# Autodesk Inventor assembly: Assembly_SIMMO_1
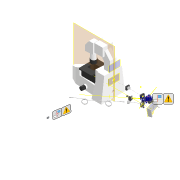
[picture p0: Inventor's stored thumbnail of the model, 180x180]
Saved by Autodesk Inventor 2022 (Build 260153000, 153)
## iProperties
Created: 2022-04-09
Part Number: Assembly_SIMMO_1
Document SubType Name: Assembly
Designer: Prakash Lab
Author: Prakash Lab
## Documents named in this file (16)
- C:\Users\PrakashLab\Documents\SIMMO\INVENTOR\Assembly_SIMMO_1.iam
- C:\Users\PrakashLab\Documents\SIMMO\INVENTOR\00_AC254-200-A-ML-Step.ipt
- C:\Users\PrakashLab\Documents\SIMMO\INVENTOR\Adapter_DMD_KM100.ipt
- C:\Users\PrakashLab\Documents\SIMMO\INVENTOR\Cover_new.ipt
- C:\Users\PrakashLab\Documents\SIMMO\INVENTOR\KM100-Solidworks.ipt
- C:\Users\PrakashLab\Documents\SIMMO\INVENTOR\Mount_new.ipt
- C:\Users\PrakashLab\Documents\SIMMO\INVENTOR\Nikon_Ti2E.ipt
- C:\Users\PrakashLab\Documents\SIMMO\INVENTOR\00_AC254-030-A-ML-Step.ipt
- C:\Users\PrakashLab\Documents\SIMMO\INVENTOR\00_AC254-075-A-ML-Step.ipt
- C:\Users\PrakashLab\Documents\SIMMO\INVENTOR\00_Beampath_v0.ipt
- C:\Users\PrakashLab\Documents\SIMMO\INVENTOR\PF10-03-P01-Solidworks.ipt
- C:\Users\PrakashLab\Documents\SIMMO\INVENTOR\00_Assembly_Axiovert.ipt
- C:\Users\PrakashLab\Documents\SIMMO\INVENTOR\00_CP33T_M-Step.ipt
- C:\Users\PrakashLab\Documents\SIMMO\INVENTOR\00_KM100-Step.ipt
- C:\Users\PrakashLab\Documents\SIMMO\INVENTOR\00_P1-305A-FC-1-Step.ipt
- C:\Users\PrakashLab\Documents\SIMMO\INVENTOR\00_PF10-03-P01-Solidworks.ipt
## Components (19 placed, 15 different names)
1. Adapter_DMD_KM100:1 — Insert:5, Mate:5, Insert:6, Mate:6
2. KM100-Solidworks:1 — Insert:6, Angle:3
3. Mount_new:1 — Mate:6
4. 00_AC254-030-A-ML-Step:1 — Insert:11, Insert:12
5. Nikon_Ti2E:1 — Mate:1, Mate:2, Mate:3, Flush:1, Flush:2, Flush:4, Mate:10, Mate:11, Angle:6
6. 00_Beampath_v0:1 — Flush:1, Flush:2, Insert:1, Insert:2, Insert:3, Angle:1, Mate:4, Angle:4, Mate:7, Mate:8, Mate:12, Insert:12, Insert:13, Insert:15
7. 00_AC254-200-A-ML-Step:1 — Insert:1
8. 00_AC254-075-A-ML-Step:1 — Insert:2, Insert:8
9. 00_AC254-075-A-ML-Step:2 — Insert:3, Insert:9
10. Cover_new:1 — Angle:1, Mate:4, Angle:2, Insert:5, Mate:5
11. PF10-03-P01-Solidworks:1 — Angle:4, Mate:7, Mate:8
12. 00_Assembly_Axiovert:1 — Flush:4, Mate:10, Mate:11, Mate:12
13. 00_CP33T_M-Step:1 — Insert:8
14. 00_CP33T_M-Step:2 — Insert:9
15. 00_KM100-Step:2 — Insert:16
16. 00_P1-305A-FC-1-Step:1 — Insert:11
17. 00_KM100-Step:3 — Insert:14, Angle:6
18. 00_PF10-03-P01-Solidworks:1 — Insert:13, Insert:14
19. 00_PF10-03-P01-Solidworks:2 — Insert:15, Insert:16
## Relationships (32: Insert 13, Mate 11, Angle 5, Flush 3)
- Mate:1: Nikon_Ti2E:1
- Mate:2: Nikon_Ti2E:1
- Mate:3: Nikon_Ti2E:1
- Flush:1: Nikon_Ti2E:1 ↔ 00_Beampath_v0:1
- Flush:2: Nikon_Ti2E:1 ↔ 00_Beampath_v0:1
- Insert:1: 00_Beampath_v0:1 ↔ 00_AC254-200-A-ML-Step:1
- Insert:2: 00_Beampath_v0:1 ↔ 00_AC254-075-A-ML-Step:1
- Insert:3: 00_Beampath_v0:1 ↔ 00_AC254-075-A-ML-Step:2
- Angle:1 (190 deg): 00_Beampath_v0:1 ↔ Cover_new:1
- Mate:4: 00_Beampath_v0:1 ↔ Cover_new:1
- Angle:2 (0 deg): Cover_new:1
- Insert:5 (5 mm): Adapter_DMD_KM100:1 ↔ Cover_new:1
- Mate:5: Adapter_DMD_KM100:1 ↔ Cover_new:1
- Insert:6 (8 mm): Adapter_DMD_KM100:1 ↔ KM100-Solidworks:1
- Mate:6 (20 mm): Adapter_DMD_KM100:1 ↔ Mount_new:1
- Angle:3 (0 deg): KM100-Solidworks:1
- Angle:4 (-53 deg): 00_Beampath_v0:1 ↔ PF10-03-P01-Solidworks:1
- Mate:7: 00_Beampath_v0:1 ↔ PF10-03-P01-Solidworks:1
- Mate:8: 00_Beampath_v0:1 ↔ PF10-03-P01-Solidworks:1
- Flush:4: Nikon_Ti2E:1 ↔ 00_Assembly_Axiovert:1
- Mate:10: Nikon_Ti2E:1 ↔ 00_Assembly_Axiovert:1
- Mate:11: Nikon_Ti2E:1 ↔ 00_Assembly_Axiovert:1
- Mate:12 (-194 mm): 00_Beampath_v0:1 ↔ 00_Assembly_Axiovert:1
- Insert:8: 00_AC254-075-A-ML-Step:1 ↔ 00_CP33T_M-Step:1
- Insert:9: 00_AC254-075-A-ML-Step:2 ↔ 00_CP33T_M-Step:2
- Insert:11 (30 mm): 00_AC254-030-A-ML-Step:1 ↔ 00_P1-305A-FC-1-Step:1
- Insert:12: 00_AC254-030-A-ML-Step:1 ↔ 00_Beampath_v0:1
- Insert:13: 00_Beampath_v0:1 ↔ 00_PF10-03-P01-Solidworks:1
- Insert:14: 00_KM100-Step:3 ↔ 00_PF10-03-P01-Solidworks:1
- Angle:6 (0 deg): Nikon_Ti2E:1 ↔ 00_KM100-Step:3
- Insert:15: 00_Beampath_v0:1 ↔ 00_PF10-03-P01-Solidworks:2
- Insert:16: 00_KM100-Step:2 ↔ 00_PF10-03-P01-Solidworks:2
